# Autodesk Inventor assembly: 42146-26
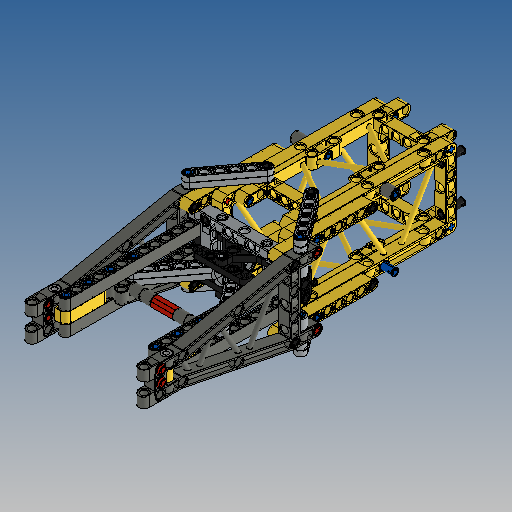
[picture p0: Inventor's stored thumbnail of the model, 512x512]
Saved by Autodesk Inventor 2025 (Build 290162010, 162A)
## iProperties
Created: 2024-11-29
Part Number: 42146-26
Material: Generisch
Document SubType Name: Assembly
Designer: hp.muther
Author: hp.muther
## Documents named in this file (23)
- D:\Inventor\Projekte\Muther\LEGO Technic\LEGO Technik - Raupenkran LR 13000 (42146)\42146-26.iam
- D:\Inventor\Projekte\Muther\LEGO Technic\LEGO Pieces\Rahmen, T-Stücke\99773-Black.ipt
- D:\Inventor\Projekte\Muther\LEGO Technic\LEGO Pieces\Verbindungselemente\48989-LtBluishGray.ipt
- D:\Inventor\Projekte\Muther\LEGO Technic\LEGO Pieces\Pin's\2780-Black.ipt
- D:\Inventor\Projekte\Muther\LEGO Technic\LEGO Pieces\Lochbalken schmal\32063-LtBluishGray.ipt
- D:\Inventor\Projekte\Muther\LEGO Technic\LEGO Pieces\Lochbalken\41239-DkBluishGray.ipt
- D:\Inventor\Projekte\Muther\LEGO Technic\LEGO Pieces\Pin's\6558-Blue.ipt
- D:\Inventor\Projekte\Muther\LEGO Technic\LEGO Pieces\Verbindungselemente\32291-DkBluishGray.ipt
- D:\Inventor\Projekte\Muther\LEGO Technic\LEGO Pieces\Rund\18654-DkBluishGray.ipt
- D:\Inventor\Projekte\Muther\LEGO Technic\LEGO Pieces\Rund\6538c-Red.ipt
- D:\Inventor\Projekte\Muther\LEGO Technic\LEGO Pieces\Achsen\99008-Tan.ipt
- D:\Inventor\Projekte\Muther\LEGO Technic\LEGO Pieces\Winkel\32140-Yellow.ipt
- D:\Inventor\Projekte\Muther\LEGO Technic\LEGO Pieces\Rahmen, T-Stücke\64178-LtBluishGray.ipt
- D:\Inventor\Projekte\Muther\LEGO Technic\LEGO Pieces\Achsen\32073-LtBluishGray.ipt
- D:\Inventor\Projekte\Muther\LEGO Technic\LEGO Pieces\Pin's\43093-Blue.ipt
- D:\Inventor\Projekte\Muther\LEGO Technic\LEGO Pieces\Rahmen, T-Stücke\79766-Yellow.ipt
- D:\Inventor\Projekte\Muther\LEGO Technic\LEGO Pieces\Rahmen, T-Stücke\79767-Yellow.ipt
- D:\Inventor\Projekte\Muther\LEGO Technic\LEGO Pieces\Verbindungselemente\63869-Black.ipt
- D:\Inventor\Projekte\Muther\LEGO Technic\LEGO Pieces\Pin's\11214-Red.ipt
- D:\Inventor\Projekte\Muther\LEGO Technic\LEGO Pieces\Lochbalken\40490-Yellow.ipt
- D:\Inventor\Projekte\Muther\LEGO Technic\LEGO Pieces\Rahmen, T-Stücke\79768-DkBluishGray.ipt
- D:\Inventor\Projekte\Muther\LEGO Technic\LEGO Pieces\Pin's\4274-Red.ipt
- D:\Inventor\Projekte\Muther\LEGO Technic\LEGO Pieces\Pin's\77765-MediumStoneGrey.ipt
## Components (111 placed, 22 different names)
1. 99773-Black:1 — Einfügen:1, Passend:1, Einfügen:2, Passend:2, Einfügen:7, Einfügen:8
2. 99773-Black:2 — Einfügen:1, Passend:1
3. 48989-LtBluishGray:1 — Einfügen:2, Passend:2, Einfügen:10, Passend:6
4. 2780-Black:1 — Einfügen:3
5. 32063-LtBluishGray:1 — Einfügen:3, Einfügen:4, Passend:3
6. 32063-LtBluishGray:2 — Einfügen:4, Passend:3, Einfügen:8, Einfügen:20
7. 2780-Black:2
8. 32063-LtBluishGray:3
9. 32063-LtBluishGray:4 — Einfügen:7, Einfügen:19
10. 99773-Black:3 — Einfügen:10, Passend:6
11. 99773-Black:4 — Einfügen:38, Passend:13, Einfügen:39, Einfügen:40
12. 41239-DkBluishGray:1 — Einfügen:11, Einfügen:12, Einfügen:13, Einfügen:14, Einfügen:20, Einfügen:30, Passend:19
13. 6558-Blue:1 — Einfügen:11
14. 6558-Blue:2 — Einfügen:12, Passend:10
15. 6558-Blue:3 — Einfügen:13, Passend:8
16. 6558-Blue:4 — Einfügen:14, Passend:12
17. 32291-DkBluishGray:1 — Einfügen:21, Einfügen:22, Einfügen:29
18. 18654-DkBluishGray:1 — Einfügen:22, Einfügen:23
19. 18654-DkBluishGray:2 — Einfügen:23, Einfügen:27
20. 6538c-Red:1 — Einfügen:27, Einfügen:28, Passend:7
21. 99008-Tan:1 — Einfügen:21
22. 32140-Yellow:1 — Einfügen:31, Passend:9, Einfügen:33, Passend:27
23. 41239-DkBluishGray:2 — Einfügen:33, Passend:11, Einfügen:76
24. 64178-LtBluishGray:1 — Einfügen:34, Einfügen:35, Einfügen:36, Einfügen:37, Einfügen:38, Passend:13, Passend:20
25. 32073-LtBluishGray:1 — Einfügen:39
26. 32073-LtBluishGray:2 — Einfügen:40
27. 2780-Black:3 — Einfügen:34
28. 2780-Black:4 — Einfügen:37
29. 2780-Black:5 — Einfügen:35
30. 2780-Black:6 — Einfügen:36
31. 41239-DkBluishGray:3 — Einfügen:19, Einfügen:29, Einfügen:31
32. 6558-Blue:5
33. 6558-Blue:6 — Passend:9
34. 6558-Blue:7
35. 6558-Blue:8 — Passend:11
36. 32291-DkBluishGray:2 — Passend:8
37. 18654-DkBluishGray:3
38. 18654-DkBluishGray:4 — Einfügen:28
39. 99008-Tan:2 — Passend:7
40. 32140-Yellow:2 — Einfügen:30, Passend:10, Einfügen:32, Passend:28
41. 41239-DkBluishGray:4 — Einfügen:32, Passend:12, Passend:20
42. 2780-Black:7 — Einfügen:43
43. 2780-Black:8 — Einfügen:44
44. 43093-Blue:1 — Einfügen:41
45. 43093-Blue:2 — Einfügen:42, Passend:14
46. 6558-Blue:9 — Einfügen:45
47. 6558-Blue:10 — Einfügen:46
48. 79766-Yellow:1 — Einfügen:49, Einfügen:50, Einfügen:51, Einfügen:52, Einfügen:53, Einfügen:54, Einfügen:56, Einfügen:69, Einfügen:63, Einfügen:68, Einfügen:62, Einfügen:55, Einfügen:75, Passend:17, Einfügen:85, Einfügen:86, Einfügen:57
49. 79767-Yellow:1 — Einfügen:47, Passend:15, Einfügen:108, Einfügen:110
50. 79767-Yellow:2 — Einfügen:48, Passend:14, Einfügen:55, Passend:16, Einfügen:96, Einfügen:97
51. 2780-Black:9 — Einfügen:51
52. 2780-Black:10 — Einfügen:52
53. 43093-Blue:3 — Einfügen:49, Passend:16
54. 43093-Blue:4 — Einfügen:50, Passend:15
55. 6558-Blue:11 — Einfügen:53
56. 6558-Blue:12 — Einfügen:54
57. 79766-Yellow:2 — Einfügen:41, Einfügen:42, Einfügen:43, Einfügen:44, Einfügen:45, Einfügen:46, Einfügen:58, Einfügen:60, Einfügen:59, Einfügen:61, Einfügen:67, Einfügen:66, Einfügen:47, Einfügen:48, Einfügen:74, Passend:18, Einfügen:83, Einfügen:84
58. 6558-Blue:13 — Einfügen:59, Einfügen:64
59. 6558-Blue:14 — Einfügen:58
60. 6558-Blue:15 — Einfügen:56
61. 6558-Blue:16 — Einfügen:57, Einfügen:65
62. 2780-Black:11 — Einfügen:63
63. 2780-Black:12 — Einfügen:62
64. 2780-Black:13 — Einfügen:60
65. 2780-Black:14 — Einfügen:61
66. 18654-DkBluishGray:5 — Einfügen:64
67. 18654-DkBluishGray:6 — Einfügen:65
68. 2780-Black:15 — Einfügen:70
69. 2780-Black:16 — Einfügen:71, Passend:17
70. 63869-Black:1 — Einfügen:70, Einfügen:71, Einfügen:75, Passend:19, Einfügen:77
71. 11214-Red:1 — Einfügen:68, Passend:22
72. 11214-Red:2 — Einfügen:69, Passend:21
73. 11214-Red:3 — Einfügen:66, Passend:24
74. 11214-Red:4 — Einfügen:67, Passend:23
75. 2780-Black:17
76. 2780-Black:18 — Passend:18
77. 63869-Black:2 — Einfügen:74, Einfügen:76, Einfügen:78
78. 32073-LtBluishGray:3 — Einfügen:78
79. 32073-LtBluishGray:4 — Einfügen:77
80. 2780-Black:19 — Einfügen:79, Passend:26
81. 40490-Yellow:1 — Einfügen:79, Einfügen:86, Passend:21
82. 2780-Black:20
83. 40490-Yellow:2 — Einfügen:85, Passend:22, Einfügen:91
84. 2780-Black:21 — Passend:25
85. 40490-Yellow:3 — Einfügen:84, Passend:24
86. 2780-Black:22
87. 40490-Yellow:4 — Einfügen:83, Passend:23, Einfügen:92
88. 79768-DkBluishGray:1 — Einfügen:87, Einfügen:88, Einfügen:92, Passend:25, Passend:27, Einfügen:94, Einfügen:95, Einfügen:107
89. 79768-DkBluishGray:2 — Einfügen:89, Einfügen:90, Einfügen:91, Passend:26, Passend:28, Einfügen:93, Einfügen:98, Einfügen:109
90. 4274-Red:1 — Einfügen:89
91. 4274-Red:2 — Einfügen:90
92. 4274-Red:3 — Einfügen:87
93. 4274-Red:4 — Einfügen:88
94. 77765-MediumStoneGrey:1 — Einfügen:94
95. 77765-MediumStoneGrey:2 — Einfügen:93
96. 6558-Blue:17 — Einfügen:95, Einfügen:102
97. 2780-Black:23 — Einfügen:96, Passend:32
98. 6558-Blue:18 — Einfügen:98, Einfügen:100
99. 2780-Black:24 — Einfügen:97, Passend:30
100. 32063-LtBluishGray:5
101. 32063-LtBluishGray:6 — Einfügen:100, Passend:30
102. 32063-LtBluishGray:7 — Einfügen:102, Passend:32
103. 32063-LtBluishGray:8
104. 6558-Blue:19 — Einfügen:107
105. 2780-Black:25 — Einfügen:108
106. 6558-Blue:20 — Einfügen:109
107. 2780-Black:26 — Einfügen:110
108. 32063-LtBluishGray:9
109. 32063-LtBluishGray:10
110. 32063-LtBluishGray:11
111. 32063-LtBluishGray:12
## Relationships (146: Insert 110, Mate 36)
- Einfügen:1 [Insert]: 99773-Black:1 ↔ 99773-Black:2
- Passend:1 [Mate]: 99773-Black:1 ↔ 99773-Black:2
- Einfügen:2 [Insert]: 99773-Black:1 ↔ 48989-LtBluishGray:1
- Passend:2 [Mate]: 99773-Black:1 ↔ 48989-LtBluishGray:1
- Einfügen:3 [Insert]: 2780-Black:1 ↔ 32063-LtBluishGray:1
- Einfügen:4 [Insert]: 32063-LtBluishGray:1 ↔ 32063-LtBluishGray:2
- Passend:3 [Mate]: 32063-LtBluishGray:1 ↔ 32063-LtBluishGray:2
- [Insert]: 2780-Black:2 ↔ 32063-LtBluishGray:3
- [Insert]: 32063-LtBluishGray:3 ↔ 32063-LtBluishGray:4
- [Mate]: 32063-LtBluishGray:3 ↔ 32063-LtBluishGray:4
- Einfügen:7 [Insert]: 99773-Black:1 ↔ 32063-LtBluishGray:4
- Einfügen:8 [Insert]: 99773-Black:1 ↔ 32063-LtBluishGray:2
- [Insert]: 99773-Black:3 ↔ 99773-Black:4
- [Mate]: 99773-Black:3 ↔ 99773-Black:4
- Einfügen:10 [Insert]: 48989-LtBluishGray:1 ↔ 99773-Black:3
- Passend:6 [Mate]: 48989-LtBluishGray:1 ↔ 99773-Black:3
- Einfügen:11 [Insert]: 41239-DkBluishGray:1 ↔ 6558-Blue:1
- Einfügen:12 [Insert]: 41239-DkBluishGray:1 ↔ 6558-Blue:2
- Einfügen:13 [Insert]: 41239-DkBluishGray:1 ↔ 6558-Blue:3
- Einfügen:14 [Insert]: 41239-DkBluishGray:1 ↔ 6558-Blue:4
- [Insert]: 41239-DkBluishGray:3 ↔ 6558-Blue:5
- [Insert]: 41239-DkBluishGray:3 ↔ 6558-Blue:6
- [Insert]: 41239-DkBluishGray:3 ↔ 6558-Blue:7
- [Insert]: 41239-DkBluishGray:3 ↔ 6558-Blue:8
- Einfügen:19 [Insert]: 32063-LtBluishGray:4 ↔ 41239-DkBluishGray:3
- Einfügen:20 [Insert]: 32063-LtBluishGray:2 ↔ 41239-DkBluishGray:1
- Einfügen:21 [Insert]: 32291-DkBluishGray:1 ↔ 99008-Tan:1
- Einfügen:22 [Insert]: 32291-DkBluishGray:1 ↔ 18654-DkBluishGray:1
- Einfügen:23 [Insert]: 18654-DkBluishGray:1 ↔ 18654-DkBluishGray:2
- [Insert]: 32291-DkBluishGray:2 ↔ 99008-Tan:2
- [Insert]: 32291-DkBluishGray:2 ↔ 18654-DkBluishGray:3
- [Insert]: 18654-DkBluishGray:3 ↔ 18654-DkBluishGray:4
- Einfügen:27 [Insert]: 18654-DkBluishGray:2 ↔ 6538c-Red:1
- Einfügen:28 [Insert]: 6538c-Red:1 ↔ 18654-DkBluishGray:4
- Passend:7 [Mate]: 6538c-Red:1 ↔ 99008-Tan:2
- Einfügen:29 [Insert]: 32291-DkBluishGray:1 ↔ 41239-DkBluishGray:3
- Passend:8 [Mate]: 6558-Blue:3 ↔ 32291-DkBluishGray:2
- Einfügen:30 [Insert]: 41239-DkBluishGray:1 ↔ 32140-Yellow:2
- Einfügen:31 [Insert]: 32140-Yellow:1 ↔ 41239-DkBluishGray:3
- Passend:9 [Mate]: 32140-Yellow:1 ↔ 6558-Blue:6
- Passend:10 [Mate]: 6558-Blue:2 ↔ 32140-Yellow:2
- Einfügen:32 [Insert]: 32140-Yellow:2 ↔ 41239-DkBluishGray:4
- Einfügen:33 [Insert]: 32140-Yellow:1 ↔ 41239-DkBluishGray:2
- Passend:11 [Mate]: 41239-DkBluishGray:2 ↔ 6558-Blue:8
- Passend:12 [Mate]: 6558-Blue:4 ↔ 41239-DkBluishGray:4
- Einfügen:34 [Insert]: 64178-LtBluishGray:1 ↔ 2780-Black:3
- Einfügen:35 [Insert]: 64178-LtBluishGray:1 ↔ 2780-Black:5
- Einfügen:36 [Insert]: 64178-LtBluishGray:1 ↔ 2780-Black:6
- Einfügen:37 [Insert]: 64178-LtBluishGray:1 ↔ 2780-Black:4
- Einfügen:38 [Insert]: 99773-Black:4 ↔ 64178-LtBluishGray:1
- Passend:13 [Mate]: 99773-Black:4 ↔ 64178-LtBluishGray:1
- Einfügen:39 [Insert] (-32 mm): 99773-Black:4 ↔ 32073-LtBluishGray:1
- Einfügen:40 [Insert] (-32 mm): 99773-Black:4 ↔ 32073-LtBluishGray:2
- Einfügen:41 [Insert]: 43093-Blue:1 ↔ 79766-Yellow:2
- Einfügen:42 [Insert]: 43093-Blue:2 ↔ 79766-Yellow:2
- Einfügen:43 [Insert]: 2780-Black:7 ↔ 79766-Yellow:2
- Einfügen:44 [Insert]: 2780-Black:8 ↔ 79766-Yellow:2
- Einfügen:45 [Insert]: 6558-Blue:9 ↔ 79766-Yellow:2
- Einfügen:46 [Insert]: 6558-Blue:10 ↔ 79766-Yellow:2
- Einfügen:47 [Insert]: 79767-Yellow:1 ↔ 79766-Yellow:2
- Einfügen:48 [Insert]: 79767-Yellow:2 ↔ 79766-Yellow:2
- Passend:14 [Mate]: 43093-Blue:2 ↔ 79767-Yellow:2
- Passend:15 [Mate]: 79767-Yellow:1 ↔ 43093-Blue:4
- Einfügen:49 [Insert]: 79766-Yellow:1 ↔ 43093-Blue:3
- Einfügen:50 [Insert]: 79766-Yellow:1 ↔ 43093-Blue:4
- Einfügen:51 [Insert]: 79766-Yellow:1 ↔ 2780-Black:9
- Einfügen:52 [Insert]: 79766-Yellow:1 ↔ 2780-Black:10
- Einfügen:53 [Insert]: 79766-Yellow:1 ↔ 6558-Blue:11
- Einfügen:54 [Insert]: 79766-Yellow:1 ↔ 6558-Blue:12
- Einfügen:55 [Insert]: 79766-Yellow:1 ↔ 79767-Yellow:2
- Passend:16 [Mate]: 79767-Yellow:2 ↔ 43093-Blue:3
- Einfügen:56 [Insert]: 79766-Yellow:1 ↔ 6558-Blue:15
- Einfügen:57 [Insert]: 79766-Yellow:1 ↔ 6558-Blue:16
- Einfügen:58 [Insert]: 79766-Yellow:2 ↔ 6558-Blue:14
- Einfügen:59 [Insert]: 79766-Yellow:2 ↔ 6558-Blue:13
- Einfügen:60 [Insert]: 79766-Yellow:2 ↔ 2780-Black:13
- Einfügen:61 [Insert]: 79766-Yellow:2 ↔ 2780-Black:14
- Einfügen:62 [Insert]: 79766-Yellow:1 ↔ 2780-Black:12
- Einfügen:63 [Insert]: 79766-Yellow:1 ↔ 2780-Black:11
- Einfügen:64 [Insert]: 6558-Blue:13 ↔ 18654-DkBluishGray:5
- Einfügen:65 [Insert]: 6558-Blue:16 ↔ 18654-DkBluishGray:6
- Einfügen:66 [Insert]: 79766-Yellow:2 ↔ 11214-Red:3
- Einfügen:67 [Insert]: 79766-Yellow:2 ↔ 11214-Red:4
- Einfügen:68 [Insert]: 79766-Yellow:1 ↔ 11214-Red:1
- Einfügen:69 [Insert]: 79766-Yellow:1 ↔ 11214-Red:2
- Einfügen:70 [Insert]: 2780-Black:15 ↔ 63869-Black:1
- Einfügen:71 [Insert]: 2780-Black:16 ↔ 63869-Black:1
- [Insert]: 2780-Black:17 ↔ 63869-Black:2
- [Insert]: 2780-Black:18 ↔ 63869-Black:2
- Einfügen:74 [Insert]: 79766-Yellow:2 ↔ 63869-Black:2
- Einfügen:75 [Insert]: 79766-Yellow:1 ↔ 63869-Black:1
- Passend:17 [Mate]: 79766-Yellow:1 ↔ 2780-Black:16
- Passend:18 [Mate]: 79766-Yellow:2 ↔ 2780-Black:18
- Einfügen:76 [Insert]: 41239-DkBluishGray:2 ↔ 63869-Black:2
- Passend:19 [Mate]: 41239-DkBluishGray:1 ↔ 63869-Black:1
- Passend:20 [Mate]: 64178-LtBluishGray:1 ↔ 41239-DkBluishGray:4
- Einfügen:77 [Insert] (-24 mm): 63869-Black:1 ↔ 32073-LtBluishGray:4
- Einfügen:78 [Insert] (-24 mm): 63869-Black:2 ↔ 32073-LtBluishGray:3
- Einfügen:79 [Insert]: 2780-Black:19 ↔ 40490-Yellow:1
- [Insert]: 2780-Black:20 ↔ 40490-Yellow:2
- [Insert]: 2780-Black:21 ↔ 40490-Yellow:3
- [Insert]: 2780-Black:22 ↔ 40490-Yellow:4
- Einfügen:83 [Insert]: 79766-Yellow:2 ↔ 40490-Yellow:4
- Einfügen:84 [Insert]: 79766-Yellow:2 ↔ 40490-Yellow:3
- Einfügen:85 [Insert]: 79766-Yellow:1 ↔ 40490-Yellow:2
- Einfügen:86 [Insert]: 79766-Yellow:1 ↔ 40490-Yellow:1
- Passend:21 [Mate]: 11214-Red:2 ↔ 40490-Yellow:1
- Passend:22 [Mate]: 11214-Red:1 ↔ 40490-Yellow:2
- Passend:23 [Mate]: 11214-Red:4 ↔ 40490-Yellow:4
- Passend:24 [Mate]: 11214-Red:3 ↔ 40490-Yellow:3
- Einfügen:87 [Insert]: 79768-DkBluishGray:1 ↔ 4274-Red:3
- Einfügen:88 [Insert]: 79768-DkBluishGray:1 ↔ 4274-Red:4
- Einfügen:89 [Insert]: 79768-DkBluishGray:2 ↔ 4274-Red:1
- Einfügen:90 [Insert]: 79768-DkBluishGray:2 ↔ 4274-Red:2
- Einfügen:91 [Insert]: 40490-Yellow:2 ↔ 79768-DkBluishGray:2
- Einfügen:92 [Insert]: 40490-Yellow:4 ↔ 79768-DkBluishGray:1
- Passend:25 [Mate]: 2780-Black:21 ↔ 79768-DkBluishGray:1
- Passend:26 [Mate]: 2780-Black:19 ↔ 79768-DkBluishGray:2
- Passend:27 [Mate]: 32140-Yellow:1 ↔ 79768-DkBluishGray:1
- Passend:28 [Mate]: 32140-Yellow:2 ↔ 79768-DkBluishGray:2
- Einfügen:93 [Insert]: 79768-DkBluishGray:2 ↔ 77765-MediumStoneGrey:2
- Einfügen:94 [Insert]: 79768-DkBluishGray:1 ↔ 77765-MediumStoneGrey:1
- Einfügen:95 [Insert]: 79768-DkBluishGray:1 ↔ 6558-Blue:17
- Einfügen:96 [Insert]: 79767-Yellow:2 ↔ 2780-Black:23
- Einfügen:97 [Insert]: 79767-Yellow:2 ↔ 2780-Black:24
- Einfügen:98 [Insert]: 79768-DkBluishGray:2 ↔ 6558-Blue:18
- [Insert]: 32063-LtBluishGray:5 ↔ 32063-LtBluishGray:6
- [Mate]: 32063-LtBluishGray:5 ↔ 32063-LtBluishGray:6
- Einfügen:100 [Insert]: 6558-Blue:18 ↔ 32063-LtBluishGray:6
- Passend:30 [Mate]: 2780-Black:24 ↔ 32063-LtBluishGray:6
- [Insert]: 32063-LtBluishGray:7 ↔ 32063-LtBluishGray:8
- [Mate]: 32063-LtBluishGray:7 ↔ 32063-LtBluishGray:8
- Einfügen:102 [Insert]: 6558-Blue:17 ↔ 32063-LtBluishGray:7
- Passend:32 [Mate]: 2780-Black:23 ↔ 32063-LtBluishGray:7
- [Insert]: 32063-LtBluishGray:9 ↔ 32063-LtBluishGray:10
- [Mate]: 32063-LtBluishGray:9 ↔ 32063-LtBluishGray:10
- [Insert]: 6558-Blue:20 ↔ 32063-LtBluishGray:10
- [Mate]: 2780-Black:26 ↔ 32063-LtBluishGray:10
- [Insert]: 32063-LtBluishGray:11 ↔ 32063-LtBluishGray:12
- [Mate]: 32063-LtBluishGray:11 ↔ 32063-LtBluishGray:12
- [Insert]: 6558-Blue:19 ↔ 32063-LtBluishGray:11
- [Mate]: 2780-Black:25 ↔ 32063-LtBluishGray:11
- Einfügen:107 [Insert]: 79768-DkBluishGray:1 ↔ 6558-Blue:19
- Einfügen:108 [Insert]: 79767-Yellow:1 ↔ 2780-Black:25
- Einfügen:109 [Insert]: 79768-DkBluishGray:2 ↔ 6558-Blue:20
- Einfügen:110 [Insert]: 79767-Yellow:1 ↔ 2780-Black:26
## Named parameters: d7_d4 = 0 mm, d8_d5 = 0 mm, d9_d6 = 0 mm, d12_d1 = 0 mm, d13_d0 = 0 mm, d20_d16 = 0 mm, d21_d17 = 0 mm, d22_d18 = 0 mm, d23_d19 = 0 mm, d29_d26 = 0 mm, d30_d27 = 0 mm, d31_d28 = 0 mm, d65_d55 = 0 mm, d66_d56 = 0 mm, d67_d57 = 0 mm, d68_d58 = 0 mm, d69_d59 = 0 mm, d70_d60 = 0 mm, d89_d87 = 0 mm, d90_d88 = 0 mm, d101_d100 = 0 mm, d102_d100 = 0 mm, d103_d100 = 0 mm, d128_d5 = 0 mm, d129_d6 = 0 mm, d132_d128_d5 = 0 mm, d133_d129_d6 = 0 mm, d136_d128_d5 = 0 mm, d137_d129_d6 = 0 mm, d138_d130 = 0 mm, d139_d131 = 0 mm, d140_d132_d128_d5 = 0 mm, d141_d133_d129_d6 = 0 mm, d142_d134 = 0 mm, d143_d135 = 0 mm
